# Autodesk Inventor assembly: controlWheelTurner
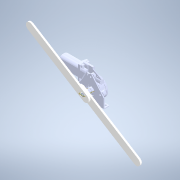
[picture p0: Inventor's stored thumbnail of the model, 180x180]
Saved by Autodesk Inventor 2020.2 (Build 242310000, 310)
## iProperties
Created: 2020-02-01
Part Number: controlWheelTurner
Document SubType Name: Assembly
Designer: robst
Author: robst
## Documents named in this file (4)
- C:\git\CAD-Development\robSteele\2020CompetitionRobot\controlWheelTurner.iam
- C:\git\CAD-Development\robSteele\2020LiftMechanism\am-2373 Snow Blower Motor Mount.ipt
- C:\git\CAD-Development\robSteele\2020BallTriggerMechanism\am-2235a Snow Blower Motor With Hex Shaft.iam
- C:\git\CAD-Development\robSteele\2020CompetitionRobot\armForTurningControlWheel.ipt
## Components (4 placed, 3 different names)
1. am-2373 Snow Blower Motor Mount:1 — Insert:1, Insert:2
2. am-2235a Snow Blower Motor With Hex Shaft:1 [sub-assembly] — Insert:1, Insert:2, Mate:1, Mate:2, Mate:3, Mate:4
3. armForTurningControlWheel:1 — Mate:1, Mate:2
4. armForTurningControlWheel:2 — Mate:3, Mate:4
## Relationships (6: Mate 4, Insert 2)
- Insert:1: am-2373 Snow Blower Motor Mount:1 ↔ am-2235a Snow Blower Motor With Hex Shaft:1
- Insert:2: am-2373 Snow Blower Motor Mount:1 ↔ am-2235a Snow Blower Motor With Hex Shaft:1
- Mate:1 (-12.7 mm): am-2235a Snow Blower Motor With Hex Shaft:1 ↔ armForTurningControlWheel:1
- Mate:2: am-2235a Snow Blower Motor With Hex Shaft:1 ↔ armForTurningControlWheel:1
- Mate:3 (-6.35 mm): am-2235a Snow Blower Motor With Hex Shaft:1 ↔ armForTurningControlWheel:2
- Mate:4: am-2235a Snow Blower Motor With Hex Shaft:1 ↔ armForTurningControlWheel:2
